# Autodesk Inventor assembly: Bird_wing_3_scaled_V1
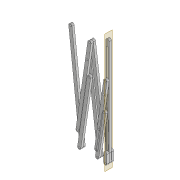
[picture p0: Inventor's stored thumbnail of the model, 180x180]
Saved by Autodesk Inventor 2022 (Build 260153000, 153)
## iProperties
Created: 2022-04-22
Part Number: Bird_wing_3_scaled_V1
Document SubType Name: Assembly
Designer: dell
Author: dell
## Documents named in this file (10)
- D:\xxxx\Uni\Part IV\MECHENG_700\Part_IV_project_CAD\Bird_skeleton_prototypes\Bird_wing_3_scaled_V1\Bird_wing_3_scaled_V1.iam
- D:\xxxx\Uni\Part IV\MECHENG_700\Part_IV_project_CAD\Bird_skeleton_prototypes\Bird_wing_3_scaled_V1\Part_6.ipt
- D:\xxxx\Uni\Part IV\MECHENG_700\Part_IV_project_CAD\Bird_skeleton_prototypes\Bird_wing_3_scaled_V1\Part_2.ipt
- D:\xxxx\Uni\Part IV\MECHENG_700\Part_IV_project_CAD\Bird_skeleton_prototypes\Bird_wing_3_scaled_V1\Part_3.ipt
- D:\xxxx\Uni\Part IV\MECHENG_700\Part_IV_project_CAD\Bird_skeleton_prototypes\Bird_wing_3_scaled_V1\Part_4.ipt
- D:\xxxx\Uni\Part IV\MECHENG_700\Part_IV_project_CAD\Bird_skeleton_prototypes\Bird_wing_3_scaled_V1\Part_5.ipt
- D:\xxxx\Uni\Part IV\MECHENG_700\Part_IV_project_CAD\Bird_skeleton_prototypes\Bird_wing_3_scaled_V1\Part_8.ipt
- D:\xxxx\Uni\Part IV\MECHENG_700\Part_IV_project_CAD\Bird_skeleton_prototypes\Bird_wing_3_scaled_V1\Part_7.ipt
- D:\xxxx\Uni\Part IV\MECHENG_700\Part_IV_project_CAD\Bird_skeleton_prototypes\Bird_wing_3_scaled_V1\Part_9.ipt
- D:\xxxx\Uni\Part IV\MECHENG_700\Part_IV_project_CAD\Bird_skeleton_prototypes\Bird_wing_3_scaled_V1\Part_10.ipt
## Components (9 placed, 9 different names)
1. Part_6:1 — Mate:1, Mate:2, Mate:3, Mate:20
2. Part_2:1 — Mate:1, Mate:2, Mate:4, Mate:5, Mate:6
3. Part_3:1 — Mate:3, Mate:4, Mate:8, Mate:10, Mate:11, Mate:20
4. Part_4:1 — Mate:5, Mate:6, Mate:7, Mate:9
5. Part_5:1 — Mate:7, Mate:8, Mate:9, Mate:14, Mate:15, Mate:16
6. Part_8:1 — Mate:10, Mate:11, Mate:12, Mate:13
7. Part_7:1 — Mate:12, Mate:13, Mate:14, Mate:19
8. Part_9:1 — Mate:15, Mate:16, Mate:17, Mate:18
9. Part_10:1 — Mate:17, Mate:18, Mate:19
## Relationships (20: Mate 20)
- Mate:1: Part_6:1 ↔ Part_2:1
- Mate:2 (0.2 mm): Part_6:1 ↔ Part_2:1
- Mate:3: Part_6:1 ↔ Part_3:1
- Mate:4: Part_2:1 ↔ Part_3:1
- Mate:5: Part_2:1 ↔ Part_4:1
- Mate:6: Part_2:1 ↔ Part_4:1
- Mate:7: Part_4:1 ↔ Part_5:1
- Mate:8: Part_3:1 ↔ Part_5:1
- Mate:9: Part_4:1 ↔ Part_5:1
- Mate:10: Part_3:1 ↔ Part_8:1
- Mate:11: Part_3:1 ↔ Part_8:1
- Mate:12: Part_8:1 ↔ Part_7:1
- Mate:13: Part_8:1 ↔ Part_7:1
- Mate:14: Part_5:1 ↔ Part_7:1
- Mate:15: Part_5:1 ↔ Part_9:1
- Mate:16: Part_5:1 ↔ Part_9:1
- Mate:17: Part_9:1 ↔ Part_10:1
- Mate:18: Part_9:1 ↔ Part_10:1
- Mate:19: Part_7:1 ↔ Part_10:1
- Mate:20: Part_6:1 ↔ Part_3:1
